# Autodesk Inventor assembly: ControllerMount
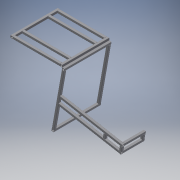
[picture p0: Inventor's stored thumbnail of the model, 180x180]
Saved by Autodesk Inventor 2016 (Build 200138000, 138)
## iProperties
Created: 2016-06-23
Part Number: ControllerMount
Document SubType Name: Assembly
Designer: cutrones
Author: cutrones
## Documents named in this file (8)
- C:\Users\cutrones\Desktop\motionbase\CAD\MotionBaseCAD\ControllerMount\ControllerMount.iam
- C:\Users\cutrones\Desktop\motionbase\CAD\MotionBaseCAD\ControllerMount\InitialVert.ipt
- C:\Users\cutrones\Desktop\motionbase\CAD\MotionBaseCAD\ControllerMount\2ndVert.ipt
- C:\Users\cutrones\Desktop\motionbase\CAD\MotionBaseCAD\ControllerMount\InitialHoriz.ipt
- C:\Users\cutrones\Desktop\motionbase\CAD\MotionBaseCAD\ControllerMount\FrontHoriz.ipt
- C:\Users\cutrones\Desktop\motionbase\CAD\MotionBaseCAD\ControllerMount\LegExtrusion.ipt
- C:\Users\cutrones\Desktop\motionbase\CAD\MotionBaseCAD\ControllerMount\LegBracing.ipt
- C:\Users\cutrones\Desktop\motionbase\CAD\MotionBaseCAD\ControllerMount\HeelBar.ipt
## Components (17 placed, 7 different names)
1. InitialVert:1 — Mate:1, Mate:2, Mate:3, Flush:1, Flush:2, Flush:5, Flush:6, Flush:7, Flush:10, Mate:8
2. 2ndVert:1 — Flush:1, Flush:2, Mate:4, Flush:3, Mate:5, Flush:4, Flush:8, Mate:6, Mate:7, Flush:9, Flush:11, Tangent:1
3. InitialHoriz:1 — Mate:4, Flush:3, Flush:5, Mate:8
4. InitialHoriz:2 — Mate:5, Flush:4, Flush:6
5. InitialHoriz:3 — Flush:7, Flush:8, Mate:6
6. InitialHoriz:4 — Mate:7, Flush:9, Flush:10
7. 2ndVert:2 — Flush:11, Tangent:1, Mate:9, Flush:12, Flush:15, Mate:11, Flush:16, Flush:19, Flush:36
8. 2ndVert:3 — Mate:10, Flush:13, Flush:14, Flush:17, Mate:12, Flush:18
9. FrontHoriz:1 — Mate:11, Flush:16, Flush:17, Mate:12, Flush:18, Flush:19, Mate:13, Flush:20, Mate:14, Flush:21
10. FrontHoriz:2 — Mate:9, Flush:12, Mate:10, Flush:13, Flush:14, Flush:15
11. LegExtrusion:1 — Mate:13, Flush:20, Flush:30, Flush:31, Mate:18, Mate:21
12. LegExtrusion:2 — Mate:14, Flush:21, Mate:15, Flush:24, Flush:25, Mate:16, Flush:26, Flush:32, Mate:19, Flush:33
13. LegBracing:2 — Mate:16, Flush:26, Flush:28, Mate:21
14. LegBracing:3 — Mate:15, Flush:24, Flush:25, Flush:28, Flush:36
15. HeelBar:1 — Flush:32, Mate:19, Flush:33, Flush:35, Mate:20
16. HeelBar:2 — Flush:30, Flush:31, Mate:18, Flush:34
17. LegBracing:4 — Flush:34, Flush:35, Mate:20
## Relationships (53: Flush 32, Mate 20, Tangent 1)
- Mate:1: InitialVert:1
- Mate:2: InitialVert:1
- Mate:3: InitialVert:1
- Flush:1: InitialVert:1 ↔ 2ndVert:1
- Flush:2: InitialVert:1 ↔ 2ndVert:1
- Mate:4: 2ndVert:1 ↔ InitialHoriz:1
- Flush:3: 2ndVert:1 ↔ InitialHoriz:1
- Mate:5: 2ndVert:1 ↔ InitialHoriz:2
- Flush:4: 2ndVert:1 ↔ InitialHoriz:2
- Flush:5 (-101.6 mm): InitialVert:1 ↔ InitialHoriz:1
- Flush:6 (101.6 mm): InitialVert:1 ↔ InitialHoriz:2
- Flush:7: InitialVert:1 ↔ InitialHoriz:3
- Flush:8: 2ndVert:1 ↔ InitialHoriz:3
- Mate:6: 2ndVert:1 ↔ InitialHoriz:3
- Mate:7: 2ndVert:1 ↔ InitialHoriz:4
- Flush:9: 2ndVert:1 ↔ InitialHoriz:4
- Flush:10: InitialVert:1 ↔ InitialHoriz:4
- Mate:8: InitialVert:1 ↔ InitialHoriz:1
- Flush:11: 2ndVert:1 ↔ 2ndVert:2
- Tangent:1: 2ndVert:1 ↔ 2ndVert:2
- Mate:9: 2ndVert:2 ↔ FrontHoriz:2
- Flush:12: 2ndVert:2 ↔ FrontHoriz:2
- Mate:10: 2ndVert:3 ↔ FrontHoriz:2
- Flush:13: 2ndVert:3 ↔ FrontHoriz:2
- Flush:14: 2ndVert:3 ↔ FrontHoriz:2
- Flush:15: 2ndVert:2 ↔ FrontHoriz:2
- Mate:11: 2ndVert:2 ↔ FrontHoriz:1
- Flush:16: 2ndVert:2 ↔ FrontHoriz:1
- Flush:17: 2ndVert:3 ↔ FrontHoriz:1
- Mate:12: 2ndVert:3 ↔ FrontHoriz:1
- Flush:18: 2ndVert:3 ↔ FrontHoriz:1
- Flush:19: 2ndVert:2 ↔ FrontHoriz:1
- Mate:13: FrontHoriz:1 ↔ LegExtrusion:1
- Flush:20: FrontHoriz:1 ↔ LegExtrusion:1
- Mate:14: FrontHoriz:1 ↔ LegExtrusion:2
- Flush:21: FrontHoriz:1 ↔ LegExtrusion:2
- Mate:15: LegExtrusion:2 ↔ LegBracing:3
- Flush:24: LegExtrusion:2 ↔ LegBracing:3
- Flush:25: LegExtrusion:2 ↔ LegBracing:3
- Mate:16: LegExtrusion:2 ↔ LegBracing:2
- Flush:26: LegExtrusion:2 ↔ LegBracing:2
- Flush:28 (177.8 mm): LegBracing:2 ↔ LegBracing:3
- Flush:30: LegExtrusion:1 ↔ HeelBar:2
- Flush:31: LegExtrusion:1 ↔ HeelBar:2
- Mate:18: LegExtrusion:1 ↔ HeelBar:2
- Flush:32: LegExtrusion:2 ↔ HeelBar:1
- Mate:19: LegExtrusion:2 ↔ HeelBar:1
- Flush:33: LegExtrusion:2 ↔ HeelBar:1
- Flush:34: HeelBar:2 ↔ LegBracing:4
- Flush:35: HeelBar:1 ↔ LegBracing:4
- Mate:20: HeelBar:1 ↔ LegBracing:4
- Mate:21: LegExtrusion:1 ↔ LegBracing:2
- Flush:36 (-279.4 mm): 2ndVert:2 ↔ LegBracing:3
